# Autodesk Inventor assembly: Final Part v2
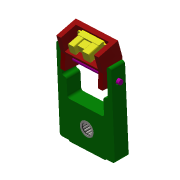
[picture p0: Inventor's stored thumbnail of the model, 180x180]
Saved by Autodesk Inventor 2018.3 (Build 223284000, 284)
## iProperties
Created: 2019-02-15
Part Number: Final Part v2
Document SubType Name: Assembly
Designer: aye06091
Mass: 123.87 g
Surface Area: 401.522 cm^2
Volume: 123.87 cm^3
Density: 1 g/cm^3
Author: aye06091
## Documents named in this file (6)
- Y:\DeSimony-R\Senior R&D\4 R&D Shared Folder\VisiStick\VisiStick (Inventor)\Physical Parts\Final Part v2.iam
- Y:\DeSimony-R\Senior R&D\4 R&D Shared Folder\VisiStick\VisiStick (Inventor)\Electronics\Sharp 2Y0A02.ipt
- Y:\DeSimony-R\Senior R&D\4 R&D Shared Folder\VisiStick\VisiStick (Inventor)\Physical Parts\Lidar Sensor Case v3.ipt
- Y:\DeSimony-R\Senior R&D\4 R&D Shared Folder\VisiStick\VisiStick (Inventor)\Physical Parts\Needle Bearing Mount.ipt
- Y:\DeSimony-R\Senior R&D\4 R&D Shared Folder\VisiStick\VisiStick (Inventor)\Physical Parts\Lidar Sensor Pivot Rod.ipt
- Y:\DeSimony-R\Senior R&D\4 R&D Shared Folder\VisiStick\VisiStick (Inventor)\Physical Parts\Needle Bearing.ipt
## Components (5 placed, 5 different names)
1. Sharp 2Y0A02:1 — Insert:1, Insert:2
2. Lidar Sensor Case v3:1 — Insert:1, Insert:2, Insert:3
3. Needle Bearing Mount:1 — Insert:3, Insert:4, Insert:5
4. Lidar Sensor Pivot Rod:1 — Insert:4
5. Needle Bearing:1 — Insert:5
## Relationships (5: Insert 5)
- Insert:1: Sharp 2Y0A02:1 ↔ Lidar Sensor Case v3:1
- Insert:2: Sharp 2Y0A02:1 ↔ Lidar Sensor Case v3:1
- Insert:3 (2.54 mm): Lidar Sensor Case v3:1 ↔ Needle Bearing Mount:1
- Insert:4 (-3.175 mm): Needle Bearing Mount:1 ↔ Lidar Sensor Pivot Rod:1
- Insert:5: Needle Bearing Mount:1 ↔ Needle Bearing:1
